# Autodesk Inventor assembly: КВ33.044.300 -  Сборка мотора Makeblock с крепление
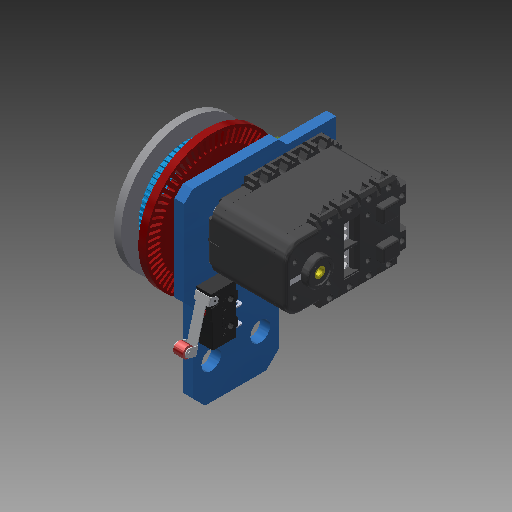
[picture p0: Inventor's stored thumbnail of the model, 512x512]
Saved by Autodesk Inventor 2019 (Build 230136000, 136)
## iProperties
Created: 2019-07-17
Part Number: КВ33.044.300 -  Сборка мотора Makeblock с крепление
Material: Типовые
Document SubType Name: Assembly
Designer: Петров Иван
Author: Петров Иван
## Documents named in this file (9)
- E:\IVAN\Kvantoriada2019\optimal_gripper\hardware\КВ33.044.500 -  Сборка сервомотора Dynamixel с крепление обратный.iam
- E:\IVAN\Kvantoriada2019\optimal_gripper\hardware\Стандартные изделия\Проставка 4 мм.ipt
- E:\IVAN\Kvantoriada2019\optimal_gripper\hardware\Стандартные изделия\Колесо оптического датчика.ipt
- E:\IVAN\Kvantoriada2019\optimal_gripper\hardware\Стандартные изделия\Шкив большой Makeblock.ipt
- E:\IVAN\Kvantoriada2019\optimal_gripper\hardware\Стандартные изделия\Сервомотор Dynamixel AX-12A\ax-12a.iam
- E:\IVAN\Kvantoriada2019\optimal_gripper\hardware\Стандартные изделия\Боковина шкива.ipt
- E:\IVAN\Kvantoriada2019\optimal_gripper\hardware\КВ33.044.501 - Деражатель мотора обратный.ipt
- E:\IVAN\Kvantoriada2019\optimal_gripper\hardware\Стандартные изделия\Датчик оптический с измененными контактами.ipt
- E:\IVAN\Kvantoriada2019\optimal_gripper\hardware\Стандартные изделия\Концевик механический\Концевик механический.ipt
## Components (8 placed, 8 different names)
1. КВ33.044.501 - Деражатель мотора обратный:1 — Совмещение:1, Совмещение:2, Совмещение:3, Совмещение:15, Совмещение:16, Совмещение:17, Совмещение:18, Совмещение:19, Совмещение:20
2. ax-12a:1 [sub-assembly] — Совмещение:1, Совмещение:2, Совмещение:3, Совмещение:4, Совмещение:5
3. Проставка 4 мм:1 — Совмещение:4, Совмещение:5, Совмещение:6, Совмещение:7, Совмещение:8
4. Колесо оптического датчика:1 — Совмещение:6, Совмещение:7, Совмещение:8, Совмещение:9, Совмещение:10, Совмещение:11
5. Шкив большой Makeblock:1 — Совмещение:9, Совмещение:10, Совмещение:11, Совмещение:12, Совмещение:13, Совмещение:14
6. Боковина шкива:1 — Совмещение:12, Совмещение:13, Совмещение:14
7. Датчик оптический с измененными контактами:1 — Совмещение:15, Совмещение:16, Совмещение:17
8. Концевик механический:1 — Совмещение:18, Совмещение:19, Совмещение:20
## Relationships (20: Mate 20)
- Совмещение:1 [Mate]: КВ33.044.501 - Деражатель мотора обратный:1 ↔ ax-12a:1
- Совмещение:2 [Mate]: КВ33.044.501 - Деражатель мотора обратный:1 ↔ ax-12a:1
- Совмещение:3 [Mate]: КВ33.044.501 - Деражатель мотора обратный:1 ↔ ax-12a:1
- Совмещение:4 [Mate]: ax-12a:1 ↔ Проставка 4 мм:1
- Совмещение:5 [Mate]: ax-12a:1 ↔ Проставка 4 мм:1
- Совмещение:6 [Mate]: Проставка 4 мм:1 ↔ Колесо оптического датчика:1
- Совмещение:7 [Mate]: Проставка 4 мм:1 ↔ Колесо оптического датчика:1
- Совмещение:8 [Mate]: Проставка 4 мм:1 ↔ Колесо оптического датчика:1
- Совмещение:9 [Mate]: Колесо оптического датчика:1 ↔ Шкив большой Makeblock:1
- Совмещение:10 [Mate]: Колесо оптического датчика:1 ↔ Шкив большой Makeblock:1
- Совмещение:11 [Mate]: Колесо оптического датчика:1 ↔ Шкив большой Makeblock:1
- Совмещение:12 [Mate]: Шкив большой Makeblock:1 ↔ Боковина шкива:1
- Совмещение:13 [Mate]: Шкив большой Makeblock:1 ↔ Боковина шкива:1
- Совмещение:14 [Mate]: Шкив большой Makeblock:1 ↔ Боковина шкива:1
- Совмещение:15 [Mate]: КВ33.044.501 - Деражатель мотора обратный:1 ↔ Датчик оптический с измененными контактами:1
- Совмещение:16 [Mate]: КВ33.044.501 - Деражатель мотора обратный:1 ↔ Датчик оптический с измененными контактами:1
- Совмещение:17 [Mate]: КВ33.044.501 - Деражатель мотора обратный:1 ↔ Датчик оптический с измененными контактами:1
- Совмещение:18 [Mate]: КВ33.044.501 - Деражатель мотора обратный:1 ↔ Концевик механический:1
- Совмещение:19 [Mate]: КВ33.044.501 - Деражатель мотора обратный:1 ↔ Концевик механический:1
- Совмещение:20 [Mate]: КВ33.044.501 - Деражатель мотора обратный:1 ↔ Концевик механический:1
